# Autodesk Inventor assembly: X-axis Idler assy
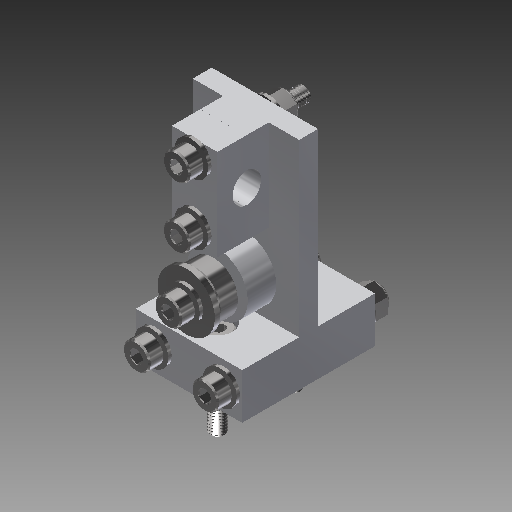
[picture p0: Inventor's stored thumbnail of the model, 512x512]
Saved by Autodesk Inventor 2018 (Build 220112000, 112)
## iProperties
Created: 2017-10-03
Part Number: X-axis Idler assy
Document SubType Name: Assembly
Designer: Gabriel Smolnycki
Author: Gabriel Smolnycki
## Documents named in this file (11)
- E:\planb\mechanics\Subassemblies\X-axis Idler 1 assy.iam
- E:\planb\mechanics\X-axis\X-axis Idler.ipt
- E:\planb\mechanics\X-axis\X-axis Rod Holder.ipt
- E:\planb\mechanics\Hardware\M4 SS Washer.ipt
- E:\planb\mechanics\Hardware\M4 SS Locknut.ipt
- E:\planb\mechanics\Hardware\M4x30 SS SHCS.ipt
- E:\planb\mechanics\X-axis\X-axis Holder Coupler.ipt
- E:\planb\mechanics\Hardware\M4x20 SS SHCS.ipt
- E:\planb\mechanics\Hardware\M4x40 SS SHCS.ipt
- E:\planb\mechanics\Hardware\M5 SS Fender Washer.ipt
- E:\planb\mechanics\Hardware\4x13 SS Ball Bearing (7804K103).ipt
## Components (30 placed, 10 different names)
1. X-axis Idler:1 — Insert:1, Insert:2, Insert:5, Insert:6, Insert:11, Insert:12, Insert:13, Insert:14, Insert:25, Insert:26
2. X-axis Rod Holder:1 — Insert:1, Insert:2, Insert:3, Insert:4
3. M4 SS Washer:1 — Insert:3, Insert:9
4. M4 SS Washer:2 — Insert:4, Insert:10
5. M4 SS Washer:3 — Insert:5, Insert:7
6. M4 SS Washer:4 — Insert:6, Insert:8
7. M4 SS Locknut:1 — Insert:7
8. M4 SS Locknut:2 — Insert:8
9. M4x30 SS SHCS:1 — Insert:9
10. M4x30 SS SHCS:2 — Insert:10
11. X-axis Holder Coupler:1 — Insert:11, Insert:12, Insert:16, Insert:19, Insert:20
12. X-axis Holder Coupler:2 — Insert:13, Insert:14, Insert:15, Insert:17, Insert:18
13. M4x20 SS SHCS:1 — Insert:16
14. M4x20 SS SHCS:2 — Insert:15
15. M4 SS Washer:5 — Insert:17, Insert:23
16. M4 SS Washer:6 — Insert:18, Insert:24
17. M4 SS Washer:7 — Insert:19, Insert:22
18. M4 SS Washer:8 — Insert:20, Insert:21
19. M4 SS Locknut:3 — Insert:21
20. M4 SS Locknut:4 — Insert:22
21. M4x40 SS SHCS:1 — Insert:23
22. M4x40 SS SHCS:2 — Insert:24
23. M4 SS Washer:9 — Insert:25, Insert:31
24. M4 SS Washer:10 — Insert:26, Insert:27
25. M4 SS Washer:11 — Insert:28, Insert:29
26. M4 SS Washer:12 — Insert:30, Insert:32
27. M5 SS Fender Washer:1 — Insert:29, Insert:30
28. 4x13 SS Ball Bearing (7804K103):1 — Insert:27, Insert:28
29. M4 SS Locknut:5 — Insert:31
30. M4x30 SS SHCS:3 — Insert:32
## Relationships (32: Insert 32)
- Insert:1: X-axis Idler:1 ↔ X-axis Rod Holder:1
- Insert:2: X-axis Idler:1 ↔ X-axis Rod Holder:1
- Insert:3: X-axis Rod Holder:1 ↔ M4 SS Washer:1
- Insert:4: X-axis Rod Holder:1 ↔ M4 SS Washer:2
- Insert:5: X-axis Idler:1 ↔ M4 SS Washer:3
- Insert:6: X-axis Idler:1 ↔ M4 SS Washer:4
- Insert:7: M4 SS Washer:3 ↔ M4 SS Locknut:1
- Insert:8: M4 SS Washer:4 ↔ M4 SS Locknut:2
- Insert:9: M4 SS Washer:1 ↔ M4x30 SS SHCS:1
- Insert:10: M4 SS Washer:2 ↔ M4x30 SS SHCS:2
- Insert:11: X-axis Idler:1 ↔ X-axis Holder Coupler:1
- Insert:12: X-axis Idler:1 ↔ X-axis Holder Coupler:1
- Insert:13: X-axis Idler:1 ↔ X-axis Holder Coupler:2
- Insert:14: X-axis Idler:1 ↔ X-axis Holder Coupler:2
- Insert:15: X-axis Holder Coupler:2 ↔ M4x20 SS SHCS:2
- Insert:16: X-axis Holder Coupler:1 ↔ M4x20 SS SHCS:1
- Insert:17: X-axis Holder Coupler:2 ↔ M4 SS Washer:5
- Insert:18: X-axis Holder Coupler:2 ↔ M4 SS Washer:6
- Insert:19: X-axis Holder Coupler:1 ↔ M4 SS Washer:7
- Insert:20: X-axis Holder Coupler:1 ↔ M4 SS Washer:8
- Insert:21: M4 SS Washer:8 ↔ M4 SS Locknut:3
- Insert:22: M4 SS Washer:7 ↔ M4 SS Locknut:4
- Insert:23: M4 SS Washer:5 ↔ M4x40 SS SHCS:1
- Insert:24: M4 SS Washer:6 ↔ M4x40 SS SHCS:2
- Insert:25: X-axis Idler:1 ↔ M4 SS Washer:9
- Insert:26: X-axis Idler:1 ↔ M4 SS Washer:10
- Insert:27: M4 SS Washer:10 ↔ 4x13 SS Ball Bearing (7804K103):1
- Insert:28: M4 SS Washer:11 ↔ 4x13 SS Ball Bearing (7804K103):1
- Insert:29: M4 SS Washer:11 ↔ M5 SS Fender Washer:1
- Insert:30: M4 SS Washer:12 ↔ M5 SS Fender Washer:1
- Insert:31: M4 SS Washer:9 ↔ M4 SS Locknut:5
- Insert:32: M4 SS Washer:12 ↔ M4x30 SS SHCS:3
